# Autodesk Inventor assembly: 射出_ベアリング3
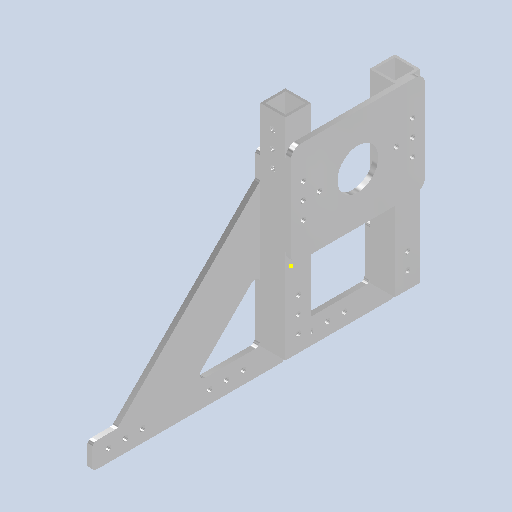
[picture p0: Inventor's stored thumbnail of the model, 512x512]
Saved by Autodesk Inventor 2023 (Build 270158000, 158)
## iProperties
Created: 2022-04-24
Part Number: 射出_ベアリング3
Document SubType Name: Assembly
Designer: yuta
Author: yuta
## Documents named in this file (6)
- C:\Users\yuta\Documents\NHK\射出_ベアリング3.iam
- C:\Users\yuta\Documents\NHK\射出_角柱10.ipt
- C:\Users\yuta\Documents\NHK\射出_角柱6.ipt
- C:\Users\yuta\Documents\NHK\射出_エンコーダー固定.ipt
- C:\Users\yuta\Documents\NHK\射出_固定2.ipt
- C:\Users\yuta\Documents\NHK\射出_固定6.ipt
## Components (5 placed, 5 different names)
1. 射出_角柱10:1 — メイト:1, メイト:2, メイト:3, メイト:7, メイト:8, メイト:9, メイト:10
2. 射出_角柱6:1 — メイト:4, メイト:5, メイト:6, メイト:11, メイト:12, メイト:13
3. 射出_エンコーダー固定:1 — メイト:1, メイト:2, メイト:3, メイト:4, メイト:5, メイト:6
4. 射出_固定2:1 — メイト:7, メイト:8, メイト:9, メイト:10
5. 射出_固定6:1 — メイト:11, メイト:12, メイト:13
## Relationships (13: Mate 13)
- メイト:1 [Mate]: 射出_角柱10:1 ↔ 射出_エンコーダー固定:1
- メイト:2 [Mate]: 射出_角柱10:1 ↔ 射出_エンコーダー固定:1
- メイト:3 [Mate]: 射出_角柱10:1 ↔ 射出_エンコーダー固定:1
- メイト:4 [Mate]: 射出_角柱6:1 ↔ 射出_エンコーダー固定:1
- メイト:5 [Mate]: 射出_角柱6:1 ↔ 射出_エンコーダー固定:1
- メイト:6 [Mate]: 射出_角柱6:1 ↔ 射出_エンコーダー固定:1
- メイト:7 [Mate]: 射出_角柱10:1 ↔ 射出_固定2:1
- メイト:8 [Mate]: 射出_角柱10:1 ↔ 射出_固定2:1
- メイト:9 [Mate]: 射出_角柱10:1 ↔ 射出_固定2:1
- メイト:10 [Mate]: 射出_角柱10:1 ↔ 射出_固定2:1
- メイト:11 [Mate]: 射出_角柱6:1 ↔ 射出_固定6:1
- メイト:12 [Mate]: 射出_角柱6:1 ↔ 射出_固定6:1
- メイト:13 [Mate]: 射出_角柱6:1 ↔ 射出_固定6:1
